# Autodesk Inventor assembly: Assembly9
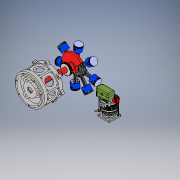
[picture p0: Inventor's stored thumbnail of the model, 180x180]
Saved by Autodesk Inventor 2018 (Build 220112000, 112)
## iProperties
Created: 2023-05-02
Part Number: Assembly9
Document SubType Name: Assembly
Designer: Habib Mohamed
Author: Habib Mohamed
## Documents named in this file (4)
- D:\Inventor\My projects\Rotary Engine\Assembly\Assembly9.iam
- D:\Inventor\My projects\Rotary Engine\Main Block (Crank Case).ipt
- D:\Inventor\My projects\Rotary Engine\Assembly\Assembly8 (Cylinder Complete Sub Assembly).iam
- D:\Inventor\My projects\Rotary Engine\Assembly\Assembly6(Piston Sub Assembly Major).iam
## Components (3 placed, 3 different names)
1. Main Block (Crank Case):1 — Mate:1
2. Assembly8 (Cylinder Complete Sub Assembly):1 [sub-assembly]
3. Assembly6(Piston Sub Assembly Major):1 [sub-assembly] — Mate:1
## Relationships (1: Mate 1)
- Mate:1: Main Block (Crank Case):1 ↔ Assembly6(Piston Sub Assembly Major):1
